# Autodesk Inventor assembly: KON_Nietmaschine_Rahmen
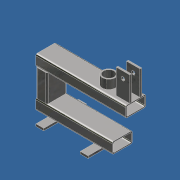
[picture p0: Inventor's stored thumbnail of the model, 180x180]
Saved by Autodesk Inventor 2019 (Build 230136000, 136)
## iProperties
Created: 2021-12-14
Part Number: KON_Nietmaschine_Rahmen
Material: Generisch
Document SubType Name: Weldment
Designer: Jonas Nebl
Weld Material: Welded Aluminum-6061
Mass: 10883.8 g
Surface Area: 5297.13 cm^2
Volume: 1386.48 cm^3
Density: 7.85 g/cm^3
Author: Jonas Nebl
## Documents named in this file (7)
- C:\Users\jonas\Documents\Inventor\Nietmaschine\KON_Nietmaschine_Rahmen.iam
- C:\Users\jonas\Documents\Inventor\Nietmaschine\DIN EN 10210-2 - 90 x 50 x 5 - 120.ipt
- C:\Users\jonas\Documents\Inventor\Nietmaschine\DIN EN 10210-2 - 90 x 50 x 5 - 400.ipt
- C:\Users\jonas\Documents\Inventor\Nietmaschine\DIN EN 10210-2 - 90 x 50 x 5 - 340.ipt
- C:\Users\jonas\Documents\Inventor\Nietmaschine\EN 10058 - 35 x 10 - 190.ipt
- C:\Users\jonas\Documents\Inventor\Nietmaschine\DIN EN 10220(2) - 57 x 5 - 100.ipt
- C:\Users\jonas\Documents\Inventor\Nietmaschine\EN 10058 - 60 x 8 - 110.ipt
## Components (8 placed, 6 different names)
1. DIN EN 10210-2 - 90 x 50 x 5 - 120:1 — Passend:1, Fluchtend:1, Fluchtend:2, Passend:2, Fluchtend:3, Fluchtend:4
2. DIN EN 10210-2 - 90 x 50 x 5 - 400:1 — Passend:1, Fluchtend:1, Fluchtend:2, Einfügen:1, Passend:5, Fluchtend:7, Fluchtend:8, Fluchtend:9, Passend:6, Fluchtend:10
3. DIN EN 10210-2 - 90 x 50 x 5 - 340:1 — Passend:2, Fluchtend:3, Fluchtend:4, Passend:3, Passend:4, Fluchtend:5, Fluchtend:6
4. EN 10058 - 35 x 10 - 190:1 — Passend:3, Fluchtend:5
5. EN 10058 - 35 x 10 - 190:2 — Passend:4, Fluchtend:6
6. DIN EN 10220(2) - 57 x 5 - 100:1 — Einfügen:1
7. EN 10058 - 60 x 8 - 110:1 — Passend:5, Fluchtend:7, Fluchtend:8
8. EN 10058 - 60 x 8 - 110:2 — Fluchtend:9, Passend:6, Fluchtend:10
## Relationships (17: Flush 10, Mate 6, Insert 1)
- Passend:1 [Mate]: DIN EN 10210-2 - 90 x 50 x 5 - 120:1 ↔ DIN EN 10210-2 - 90 x 50 x 5 - 400:1
- Fluchtend:1 [Flush]: DIN EN 10210-2 - 90 x 50 x 5 - 120:1 ↔ DIN EN 10210-2 - 90 x 50 x 5 - 400:1
- Fluchtend:2 [Flush]: DIN EN 10210-2 - 90 x 50 x 5 - 120:1 ↔ DIN EN 10210-2 - 90 x 50 x 5 - 400:1
- Passend:2 [Mate]: DIN EN 10210-2 - 90 x 50 x 5 - 120:1 ↔ DIN EN 10210-2 - 90 x 50 x 5 - 340:1
- Fluchtend:3 [Flush]: DIN EN 10210-2 - 90 x 50 x 5 - 120:1 ↔ DIN EN 10210-2 - 90 x 50 x 5 - 340:1
- Fluchtend:4 [Flush]: DIN EN 10210-2 - 90 x 50 x 5 - 120:1 ↔ DIN EN 10210-2 - 90 x 50 x 5 - 340:1
- Passend:3 [Mate]: DIN EN 10210-2 - 90 x 50 x 5 - 340:1 ↔ EN 10058 - 35 x 10 - 190:1
- Passend:4 [Mate]: DIN EN 10210-2 - 90 x 50 x 5 - 340:1 ↔ EN 10058 - 35 x 10 - 190:2
- Fluchtend:5 [Flush] (50 mm): DIN EN 10210-2 - 90 x 50 x 5 - 340:1 ↔ EN 10058 - 35 x 10 - 190:1
- Fluchtend:6 [Flush] (50 mm): DIN EN 10210-2 - 90 x 50 x 5 - 340:1 ↔ EN 10058 - 35 x 10 - 190:2
- Einfügen:1 [Insert] (-15 mm): DIN EN 10210-2 - 90 x 50 x 5 - 400:1 ↔ DIN EN 10220(2) - 57 x 5 - 100:1
- Passend:5 [Mate]: DIN EN 10210-2 - 90 x 50 x 5 - 400:1 ↔ EN 10058 - 60 x 8 - 110:1
- Fluchtend:7 [Flush] (18 mm): DIN EN 10210-2 - 90 x 50 x 5 - 400:1 ↔ EN 10058 - 60 x 8 - 110:1
- Fluchtend:8 [Flush]: DIN EN 10210-2 - 90 x 50 x 5 - 400:1 ↔ EN 10058 - 60 x 8 - 110:1
- Fluchtend:9 [Flush]: DIN EN 10210-2 - 90 x 50 x 5 - 400:1 ↔ EN 10058 - 60 x 8 - 110:2
- Passend:6 [Mate]: DIN EN 10210-2 - 90 x 50 x 5 - 400:1 ↔ EN 10058 - 60 x 8 - 110:2
- Fluchtend:10 [Flush] (18 mm): DIN EN 10210-2 - 90 x 50 x 5 - 400:1 ↔ EN 10058 - 60 x 8 - 110:2
